# Autodesk Inventor assembly: Dual Wheel Shooter MASTER
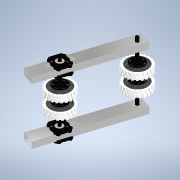
[picture p0: Inventor's stored thumbnail of the model, 180x180]
Saved by Autodesk Inventor 2020 (Build 240168000, 168)
## iProperties
Created: 2020-01-16
Part Number: Dual Wheel Shooter MASTER
Document SubType Name: Assembly
Designer: autum
Author: autum
## Documents named in this file (6)
- C:\Users\autum\Google Drive\Iron Riders 4180 (Roosevelt Robotics)\2019-2020\Build_Design\Robot 2020\Manipulators\Dual Wheel Shooter\Dual Wheel Shooter MASTER.iam
- C:\Users\autum\Google Drive\Iron Riders 4180 (Roosevelt Robotics)\2019-2020\Build_Design\Robot 2020\Manipulators\Dual Wheel Shooter\Frame.ipt
- C:\Users\autum\Google Drive\Iron Riders 4180 (Roosevelt Robotics)\2019-2020\Build_Design\Robot 2020\Manipulators\Dual Wheel Shooter\0_500_Hex_ID_x_1_125_OD_x_0_313_WD_Flanged_Bearing_v2_217-3875.ipt
- C:\Users\autum\Google Drive\Iron Riders 4180 (Roosevelt Robotics)\2019-2020\Build_Design\Robot 2020\Manipulators\Dual Wheel Shooter\VersaBlock_V2_217-6111.ipt
- C:\Users\autum\Google Drive\Iron Riders 4180 (Roosevelt Robotics)\2019-2020\Build_Design\Robot 2020\Manipulators\Dual Wheel Shooter\Hex Shaft.ipt
- C:\Users\autum\Google Drive\Iron Riders 4180 (Roosevelt Robotics)\2019-2020\Build_Design\Robot 2020\Manipulators\Dual Wheel Shooter\am-2256 4 in HiGrip Wheel.iam
## Components (18 placed, 5 different names)
1. Frame:1 — Flush:1, Mate:1, Flush:2, Insert:1, Mate:2, Mate:3, Mate:4, Mate:5, Mate:22, Mate:28
2. Frame:2 — Flush:1, Mate:1, Flush:2, Insert:2, Mate:6, Mate:7, Mate:8, Mate:9, Flush:3, Mate:25, Mate:31
3. 0_500_Hex_ID_x_1_125_OD_x_0_313_WD_Flanged_Bearing_v2_217-3875:1 — Insert:1
4. 0_500_Hex_ID_x_1_125_OD_x_0_313_WD_Flanged_Bearing_v2_217-3875:2 — Insert:2, Mate:10, Mate:11
5. 0_500_Hex_ID_x_1_125_OD_x_0_313_WD_Flanged_Bearing_v2_217-3875:3 — Insert:6, Mate:19
6. 0_500_Hex_ID_x_1_125_OD_x_0_313_WD_Flanged_Bearing_v2_217-3875:4 — Insert:5, Mate:18
7. 0_500_Hex_ID_x_1_125_OD_x_0_313_WD_Flanged_Bearing_v2_217-3875:5 — Insert:4, Mate:14, Mate:15
8. 0_500_Hex_ID_x_1_125_OD_x_0_313_WD_Flanged_Bearing_v2_217-3875:6 — Insert:3, Mate:16, Mate:17
9. VersaBlock_V2_217-6111:1 — Insert:6, Mate:4, Mate:5, Flush:4
10. VersaBlock_V2_217-6111:2 — Insert:5, Mate:2, Mate:3
11. VersaBlock_V2_217-6111:3 — Insert:4, Mate:6, Mate:7
12. VersaBlock_V2_217-6111:4 — Insert:3, Mate:8, Mate:9
13. Hex Shaft:1 — Mate:14, Mate:15, Mate:16, Mate:17, Mate:18, Mate:19, Flush:4, Mate:26, Mate:27, Mate:29, Mate:30
14. Hex Shaft:2 — Mate:10, Mate:11, Flush:3, Mate:20, Mate:21, Mate:23, Mate:24
15. am-2256 4 in HiGrip Wheel:1 [sub-assembly] — Mate:23, Mate:24, Mate:25
16. am-2256 4 in HiGrip Wheel:2 [sub-assembly] — Mate:26, Mate:27, Mate:28
17. am-2256 4 in HiGrip Wheel:3 [sub-assembly] — Mate:20, Mate:21, Mate:22
18. am-2256 4 in HiGrip Wheel:4 [sub-assembly] — Mate:29, Mate:30, Mate:31
## Relationships (39: Mate 29, Insert 6, Flush 4)
- Flush:1: Frame:1 ↔ Frame:2
- Mate:1 (203.2 mm): Frame:1 ↔ Frame:2
- Flush:2: Frame:1 ↔ Frame:2
- Insert:1: Frame:1 ↔ 0_500_Hex_ID_x_1_125_OD_x_0_313_WD_Flanged_Bearing_v2_217-3875:1
- Insert:2: Frame:2 ↔ 0_500_Hex_ID_x_1_125_OD_x_0_313_WD_Flanged_Bearing_v2_217-3875:2
- Insert:3: 0_500_Hex_ID_x_1_125_OD_x_0_313_WD_Flanged_Bearing_v2_217-3875:6 ↔ VersaBlock_V2_217-6111:4
- Insert:4: 0_500_Hex_ID_x_1_125_OD_x_0_313_WD_Flanged_Bearing_v2_217-3875:5 ↔ VersaBlock_V2_217-6111:3
- Insert:5: 0_500_Hex_ID_x_1_125_OD_x_0_313_WD_Flanged_Bearing_v2_217-3875:4 ↔ VersaBlock_V2_217-6111:2
- Insert:6: 0_500_Hex_ID_x_1_125_OD_x_0_313_WD_Flanged_Bearing_v2_217-3875:3 ↔ VersaBlock_V2_217-6111:1
- Mate:2: Frame:1 ↔ VersaBlock_V2_217-6111:2
- Mate:3: Frame:1 ↔ VersaBlock_V2_217-6111:2
- Mate:4: Frame:1 ↔ VersaBlock_V2_217-6111:1
- Mate:5: Frame:1 ↔ VersaBlock_V2_217-6111:1
- Mate:6: Frame:2 ↔ VersaBlock_V2_217-6111:3
- Mate:7: Frame:2 ↔ VersaBlock_V2_217-6111:3
- Mate:8: Frame:2 ↔ VersaBlock_V2_217-6111:4
- Mate:9: Frame:2 ↔ VersaBlock_V2_217-6111:4
- Mate:10: 0_500_Hex_ID_x_1_125_OD_x_0_313_WD_Flanged_Bearing_v2_217-3875:2 ↔ Hex Shaft:2
- Mate:11: 0_500_Hex_ID_x_1_125_OD_x_0_313_WD_Flanged_Bearing_v2_217-3875:2 ↔ Hex Shaft:2
- Flush:3 (-12.7 mm): Frame:2 ↔ Hex Shaft:2
- Mate:14: 0_500_Hex_ID_x_1_125_OD_x_0_313_WD_Flanged_Bearing_v2_217-3875:5 ↔ Hex Shaft:1
- Mate:15: 0_500_Hex_ID_x_1_125_OD_x_0_313_WD_Flanged_Bearing_v2_217-3875:5 ↔ Hex Shaft:1
- Mate:16: 0_500_Hex_ID_x_1_125_OD_x_0_313_WD_Flanged_Bearing_v2_217-3875:6 ↔ Hex Shaft:1
- Mate:17: 0_500_Hex_ID_x_1_125_OD_x_0_313_WD_Flanged_Bearing_v2_217-3875:6 ↔ Hex Shaft:1
- Mate:18: 0_500_Hex_ID_x_1_125_OD_x_0_313_WD_Flanged_Bearing_v2_217-3875:4 ↔ Hex Shaft:1
- Mate:19: 0_500_Hex_ID_x_1_125_OD_x_0_313_WD_Flanged_Bearing_v2_217-3875:3 ↔ Hex Shaft:1
- Flush:4 (-7.62 mm): VersaBlock_V2_217-6111:1 ↔ Hex Shaft:1
- Mate:20: Hex Shaft:2 ↔ am-2256 4 in HiGrip Wheel:3
- Mate:21: Hex Shaft:2 ↔ am-2256 4 in HiGrip Wheel:3
- Mate:22 (50.8 mm): Frame:1 ↔ am-2256 4 in HiGrip Wheel:3
- Mate:23: Hex Shaft:2 ↔ am-2256 4 in HiGrip Wheel:1
- Mate:24: Hex Shaft:2 ↔ am-2256 4 in HiGrip Wheel:1
- Mate:25 (50.8 mm): Frame:2 ↔ am-2256 4 in HiGrip Wheel:1
- Mate:26: Hex Shaft:1 ↔ am-2256 4 in HiGrip Wheel:2
- Mate:27: Hex Shaft:1 ↔ am-2256 4 in HiGrip Wheel:2
- Mate:28 (50.8 mm): Frame:1 ↔ am-2256 4 in HiGrip Wheel:2
- Mate:29: Hex Shaft:1 ↔ am-2256 4 in HiGrip Wheel:4
- Mate:30: Hex Shaft:1 ↔ am-2256 4 in HiGrip Wheel:4
- Mate:31 (50.8 mm): Frame:2 ↔ am-2256 4 in HiGrip Wheel:4
